# Autodesk Inventor assembly: Updated Frame
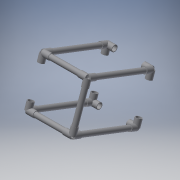
[picture p0: Inventor's stored thumbnail of the model, 180x180]
Saved by Autodesk Inventor 2016 (Build 200138000, 138)
## iProperties
Created: 2017-09-21
Part Number: Updated Frame
Document SubType Name: Assembly
Designer: Student
Author: Student
## Documents named in this file (4)
- C:\Users\Student\Documents\Derek Code and Projects\Updated ROV model\Updated Frame.iam
- C:\Users\Student\Documents\Derek Code and Projects\CodeBenderCode-master\ROV PVC Pipes\pvc pipe 1in 1ft 1.ipt
- C:\Users\Student\Documents\Derek Code and Projects\CodeBenderCode-master\ROV PVC Pipes\pvc 1in 3 way elbow.ipt
- C:\Users\Student\Documents\Derek Code and Projects\CodeBenderCode-master\ROV PVC Pipes\pvc pipe 1in 1.ipt
## Components (15 placed, 3 different names)
1. pvc pipe 1in 1ft 1:2 — Mate:6, Mate:7, Mate:18, Mate:19
2. pvc pipe 1in 1ft 1:3 — Mate:4, Mate:5, Mate:20
3. pvc pipe 1in 1ft 1:4 — Mate:1, Mate:8, Mate:16, Mate:17
4. pvc 1in 3 way elbow:1 — Mate:1, Mate:9, Mate:12, Mate:16, Mate:24
5. pvc 1in 3 way elbow:2 — Mate:7, Mate:8, Mate:13, Mate:17, Mate:18, Mate:21
6. pvc 1in 3 way elbow:3 — Mate:5, Mate:6, Mate:11, Mate:19, Mate:20, Mate:22
7. pvc 1in 3 way elbow:4 — Mate:4, Mate:9, Mate:10, Mate:23
8. pvc pipe 1in 1:1 — Mate:13, Mate:21, Mate:30
9. pvc pipe 1in 1:2 — Mate:11, Mate:15, Mate:22, Mate:27
10. pvc pipe 1in 1:3 — Mate:12, Mate:24, Mate:28
11. pvc pipe 1in 1:4 — Mate:10, Mate:14, Mate:23, Mate:26
12. pvc 1in 3 way elbow:5 — Mate:28, Mate:29, Mate:31
13. pvc 1in 3 way elbow:6 — Mate:30, Mate:31
14. pvc 1in 3 way elbow:7 — Mate:15, Mate:25, Mate:27
15. pvc 1in 3 way elbow:8 — Mate:14, Mate:25, Mate:26, Mate:29
## Relationships (29: Mate 29)
- Mate:1: pvc pipe 1in 1ft 1:4 ↔ pvc 1in 3 way elbow:1
- Mate:4: pvc pipe 1in 1ft 1:3 ↔ pvc 1in 3 way elbow:4
- Mate:5: pvc pipe 1in 1ft 1:3 ↔ pvc 1in 3 way elbow:3
- Mate:6: pvc pipe 1in 1ft 1:2 ↔ pvc 1in 3 way elbow:3
- Mate:7: pvc pipe 1in 1ft 1:2 ↔ pvc 1in 3 way elbow:2
- Mate:8: pvc pipe 1in 1ft 1:4 ↔ pvc 1in 3 way elbow:2
- Mate:9: pvc 1in 3 way elbow:1 ↔ pvc 1in 3 way elbow:4
- Mate:10: pvc 1in 3 way elbow:4 ↔ pvc pipe 1in 1:4
- Mate:11: pvc 1in 3 way elbow:3 ↔ pvc pipe 1in 1:2
- Mate:12: pvc 1in 3 way elbow:1 ↔ pvc pipe 1in 1:3
- Mate:13: pvc 1in 3 way elbow:2 ↔ pvc pipe 1in 1:1
- Mate:14: pvc pipe 1in 1:4 ↔ pvc 1in 3 way elbow:8
- Mate:15: pvc pipe 1in 1:2 ↔ pvc 1in 3 way elbow:7
- Mate:16: pvc pipe 1in 1ft 1:4 ↔ pvc 1in 3 way elbow:1
- Mate:17: pvc pipe 1in 1ft 1:4 ↔ pvc 1in 3 way elbow:2
- Mate:18: pvc pipe 1in 1ft 1:2 ↔ pvc 1in 3 way elbow:2
- Mate:19: pvc pipe 1in 1ft 1:2 ↔ pvc 1in 3 way elbow:3
- Mate:20: pvc pipe 1in 1ft 1:3 ↔ pvc 1in 3 way elbow:3
- Mate:21: pvc 1in 3 way elbow:2 ↔ pvc pipe 1in 1:1
- Mate:22: pvc 1in 3 way elbow:3 ↔ pvc pipe 1in 1:2
- Mate:23: pvc 1in 3 way elbow:4 ↔ pvc pipe 1in 1:4
- Mate:24: pvc 1in 3 way elbow:1 ↔ pvc pipe 1in 1:3
- Mate:25: pvc 1in 3 way elbow:7 ↔ pvc 1in 3 way elbow:8
- Mate:26: pvc pipe 1in 1:4 ↔ pvc 1in 3 way elbow:8
- Mate:27: pvc pipe 1in 1:2 ↔ pvc 1in 3 way elbow:7
- Mate:28: pvc pipe 1in 1:3 ↔ pvc 1in 3 way elbow:5
- Mate:29: pvc 1in 3 way elbow:5 ↔ pvc 1in 3 way elbow:8
- Mate:30: pvc pipe 1in 1:1 ↔ pvc 1in 3 way elbow:6
- Mate:31: pvc 1in 3 way elbow:5 ↔ pvc 1in 3 way elbow:6
